# Autodesk Inventor assembly: Tilter
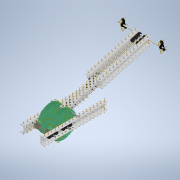
[picture p0: Inventor's stored thumbnail of the model, 180x180]
Saved by Autodesk Inventor 2020 (Build 240168000, 168)
## iProperties
Created: 2019-11-13
Part Number: Tilter
Document SubType Name: Assembly
Designer: Alex Zaccardelli
Author: Alex Zaccardelli
## Documents named in this file (11)
- D:\TrayBotCAD\Tilter.iam
- D:\TrayBotCAD\SIGBotsCADLibrary-20191023T040826Z-001\SIGBotsCADLibrary\SIGBotsCADLibrary\Structure\C-Channel 2 x 18 (aluminum).ipt
- D:\TrayBotCAD\SIGBotsCADLibrary-20191023T040826Z-001\SIGBotsCADLibrary\SIGBotsCADLibrary\Motion\Gear HS 84 tooth (fixed).iam
- D:\TrayBotCAD\SIGBotsCADLibrary-20191023T040826Z-001\SIGBotsCADLibrary\SIGBotsCADLibrary\Motion\Pillow Block.ipt
- D:\TrayBotCAD\SIGBotsCADLibrary-20191023T040826Z-001\SIGBotsCADLibrary\SIGBotsCADLibrary\Structure\C-Channel 2 x 15 (aluminum).ipt
- D:\TrayBotCAD\SIGBotsCADLibrary-20191023T040826Z-001\SIGBotsCADLibrary\SIGBotsCADLibrary\Structure\C-Channel 2 x 10 (aluminum).ipt
- D:\TrayBotCAD\SIGBotsCADLibrary-20191023T040826Z-001\SIGBotsCADLibrary\SIGBotsCADLibrary\Motion\Bearing Block.ipt
- D:\TrayBotCAD\SIGBotsCADLibrary-20191023T040826Z-001\SIGBotsCADLibrary\SIGBotsCADLibrary\Structure\Bolt 2.0 inch.ipt
- D:\TrayBotCAD\SIGBotsCADLibrary-20191023T040826Z-001\SIGBotsCADLibrary\SIGBotsCADLibrary\Motion\Shaft 4 inch.ipt
- D:\TrayBotCAD\SIGBotsCADLibrary-20191023T040826Z-001\SIGBotsCADLibrary\SIGBotsCADLibrary\Motion\Shaft 6.0 inch.ipt
- D:\TrayBotCAD\SIGBotsCADLibrary-20191023T040826Z-001\SIGBotsCADLibrary\SIGBotsCADLibrary\Motion\Gear HS 12 tooth.ipt
## Components (27 placed, 10 different names)
1. C-Channel 2 x 18 (aluminum):1
2. C-Channel 2 x 18 (aluminum):2
3. Gear HS 84 tooth (fixed):1 [sub-assembly]
4. Gear HS 84 tooth (fixed):2 [sub-assembly]
5. Pillow Block:1 — Angle:3
6. Pillow Block:2 — Angle:2
7. C-Channel 2 x 15 (aluminum):1 — Mate:53, Angle:2, Angle:4
8. C-Channel 2 x 15 (aluminum):2 — Angle:3
9. C-Channel 2 x 10 (aluminum):1 — Mate:53, Angle:4
10. Bearing Block:1 — Mate:54
11. Bearing Block:2
12. Bearing Block:3
13. Bolt 2.0 inch:1 — Mate:54
14. Bearing Block:4
15. Bearing Block:5
16. Shaft 4 inch:1
17. Shaft 4 inch:2
18. Shaft 4 inch:3
19. Bearing Block:6
20. Bearing Block:7
21. Shaft 6.0 inch:1
22. Bearing Block:8
23. Bearing Block:9
24. Gear HS 12 tooth:1
25. Gear HS 12 tooth:2
26. Bearing Block:10
27. Bearing Block:11
## Relationships (63: Mate 54, Flush 5, Angle 4)
- [Mate] (4.7498 mm): C-Channel 2 x 18 (aluminum):1 ↔ Gear HS 84 tooth (fixed):1
- [Mate]: C-Channel 2 x 18 (aluminum):1 ↔ Gear HS 84 tooth (fixed):1
- [Mate] (4.7498 mm): C-Channel 2 x 18 (aluminum):2 ↔ Gear HS 84 tooth (fixed):2
- [Mate]: Gear HS 84 tooth (fixed):1 ↔ Gear HS 84 tooth (fixed):2
- [Angle] (0 deg): C-Channel 2 x 15 (aluminum):1 ↔ C-Channel 2 x 15 (aluminum):2
- [Mate]: Pillow Block:2 ↔ C-Channel 2 x 15 (aluminum):1
- [Mate] (25.4 mm): C-Channel 2 x 15 (aluminum):1 ↔ C-Channel 2 x 15 (aluminum):2
- [Mate]: Pillow Block:1 ↔ C-Channel 2 x 15 (aluminum):2
- [Mate] (52.5907 mm): Pillow Block:1 ↔ C-Channel 2 x 15 (aluminum):2
- [Mate]: Gear HS 84 tooth (fixed):2 ↔ C-Channel 2 x 10 (aluminum):1
- [Mate]: Gear HS 84 tooth (fixed):2 ↔ C-Channel 2 x 10 (aluminum):1
- [Mate]: Gear HS 84 tooth (fixed):1 ↔ C-Channel 2 x 10 (aluminum):1
- [Mate]: C-Channel 2 x 15 (aluminum):2 ↔ C-Channel 2 x 10 (aluminum):1
- [Mate]: C-Channel 2 x 10 (aluminum):1 ↔ Bearing Block:1
- [Mate]: C-Channel 2 x 15 (aluminum):1 ↔ Bearing Block:1
- [Mate]: C-Channel 2 x 10 (aluminum):1 ↔ Bearing Block:1
- [Mate]: C-Channel 2 x 10 (aluminum):1 ↔ Bearing Block:2
- [Mate]: C-Channel 2 x 15 (aluminum):2 ↔ Bearing Block:2
- [Mate]: C-Channel 2 x 10 (aluminum):1 ↔ Bearing Block:2
- [Mate]: C-Channel 2 x 15 (aluminum):2 ↔ Bearing Block:3
- [Mate]: C-Channel 2 x 10 (aluminum):1 ↔ Bearing Block:3
- [Mate]: C-Channel 2 x 15 (aluminum):2 ↔ Bearing Block:3
- [Mate]: Bearing Block:2 ↔ Bolt 2.0 inch:1
- [Mate]: C-Channel 2 x 18 (aluminum):1 ↔ Bearing Block:4
- [Mate]: C-Channel 2 x 18 (aluminum):1 ↔ Bearing Block:4
- [Mate]: C-Channel 2 x 18 (aluminum):1 ↔ Bearing Block:4
- [Mate]: C-Channel 2 x 18 (aluminum):2 ↔ Bearing Block:5
- [Mate]: C-Channel 2 x 18 (aluminum):2 ↔ Bearing Block:5
- [Mate]: C-Channel 2 x 18 (aluminum):2 ↔ Bearing Block:5
- [Mate]: Bearing Block:4 ↔ Shaft 4 inch:1
- [Flush] (-12.7 mm): Bearing Block:5 ↔ Shaft 4 inch:1
- [Mate]: Gear HS 84 tooth (fixed):1 ↔ Shaft 4 inch:3
- [Flush] (-25.4 mm): Gear HS 84 tooth (fixed):1 ↔ Shaft 4 inch:3
- [Mate]: C-Channel 2 x 10 (aluminum):1 ↔ Bearing Block:6
- [Mate]: Shaft 4 inch:3 ↔ Bearing Block:6
- [Mate]: C-Channel 2 x 10 (aluminum):1 ↔ Bearing Block:6
- [Mate]: C-Channel 2 x 10 (aluminum):1 ↔ Bearing Block:7
- [Mate]: Bearing Block:6 ↔ Bearing Block:7
- [Mate]: Bearing Block:6 ↔ Bearing Block:7
- [Mate]: Pillow Block:1 ↔ Shaft 6.0 inch:1
- [Mate] (-3.3909 mm): Pillow Block:1 ↔ Shaft 6.0 inch:1
- [Mate]: C-Channel 2 x 15 (aluminum):2 ↔ Bearing Block:8
- [Mate]: C-Channel 2 x 15 (aluminum):2 ↔ Bearing Block:8
- [Mate]: Shaft 6.0 inch:1 ↔ Bearing Block:8
- [Mate]: C-Channel 2 x 15 (aluminum):1 ↔ Bearing Block:9
- [Mate]: Bearing Block:8 ↔ Bearing Block:9
- [Mate]: Bearing Block:8 ↔ Bearing Block:9
- [Flush]: Gear HS 84 tooth (fixed):2 ↔ Gear HS 12 tooth:1
- [Mate]: C-Channel 2 x 18 (aluminum):2 ↔ Gear HS 12 tooth:1
- [Mate]: C-Channel 2 x 18 (aluminum):1 ↔ Gear HS 12 tooth:2
- [Flush]: Gear HS 84 tooth (fixed):1 ↔ Gear HS 12 tooth:2
- [Mate]: C-Channel 2 x 18 (aluminum):2 ↔ Bearing Block:10
- [Mate]: C-Channel 2 x 18 (aluminum):2 ↔ Bearing Block:10
- [Mate]: Shaft 4 inch:2 ↔ Gear HS 12 tooth:2
- [Mate]: C-Channel 2 x 18 (aluminum):1 ↔ Bearing Block:11
- [Mate]: Shaft 4 inch:2 ↔ Bearing Block:11
- [Mate]: C-Channel 2 x 18 (aluminum):1 ↔ Bearing Block:11
- [Flush] (-7.62 mm): Shaft 4 inch:2 ↔ Bearing Block:11
- Mate:53: C-Channel 2 x 15 (aluminum):1 ↔ C-Channel 2 x 10 (aluminum):1
- Mate:54: Bearing Block:1 ↔ Bolt 2.0 inch:1
- Angle:2 (0 deg): Pillow Block:2 ↔ C-Channel 2 x 15 (aluminum):1
- Angle:3 (0 deg): Pillow Block:1 ↔ C-Channel 2 x 15 (aluminum):2
- Angle:4 (0 deg): C-Channel 2 x 15 (aluminum):1 ↔ C-Channel 2 x 10 (aluminum):1
